# Autodesk Inventor assembly: MotorEsOrsoHajtas
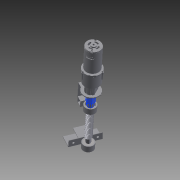
[picture p0: Inventor's stored thumbnail of the model, 180x180]
Saved by Autodesk Inventor 2015 SP1 (Build 190203100, 203)
## iProperties
Created: 2014-10-20
Part Number: MotorEsOrsoHajtas
Document SubType Name: Assembly
Designer: laca
Author: laca
## Documents named in this file (8)
- C:\Users\laca\Desktop\RobotMechanika\MotorEsOrsoHajtas.iam
- C:\Users\laca\Desktop\RobotMechanika\MotorTartoElso.ipt
- C:\Users\laca\Desktop\RobotMechanika\HatsoTartoJobb.ipt
- C:\Users\laca\Desktop\RobotMechanika\AnyaKicsi.ipt
- C:\Users\laca\Desktop\RobotMechanika\Csapagy6900.ipt
- C:\Users\laca\Desktop\RobotMechanika\Biztositek15mm.ipt
- C:\Users\laca\Desktop\RobotMechanika\Motor.iam
- C:\Users\laca\Desktop\RobotMechanika\Worm1.ipt
## Components (9 placed, 7 different names)
1. MotorTartoElso:1 — Rigid:1, Insert:5, Insert:6
2. HatsoTartoJobb:1 — Rotational:3
3. AnyaKicsi:1 — Rigid:3, Rigid:4, Cylindrical:7
4. Csapagy6900:1 — Rotational:3, Rigid:5
5. Csapagy6900:2 — Rigid:1, Cylindrical:6
6. Biztositek15mm:1 — Rigid:3, Cylindrical:5
7. Biztositek15mm:2 — Rigid:4, Cylindrical:4
8. Motor:1 [sub-assembly] — Insert:5, Cylindrical:4, Insert:6
9. Worm:2 — Rigid:5, Cylindrical:5, Cylindrical:6, Cylindrical:7
## Relationships (11: WeldJoint 4, CylindricalJoint 4, Insert 2, RevoluteJoint 1)
- Rotational:3 [RevoluteJoint]: HatsoTartoJobb:1 ↔ Csapagy6900:1
- Rigid:1 [WeldJoint]: MotorTartoElso:1 ↔ Csapagy6900:2
- Rigid:3 [WeldJoint]: AnyaKicsi:1 ↔ Biztositek15mm:1
- Rigid:4 [WeldJoint]: AnyaKicsi:1 ↔ Biztositek15mm:2
- Insert:5: MotorTartoElso:1 ↔ Motor:1
- Cylindrical:4: Biztositek15mm:2 ↔ Motor:1
- Insert:6: MotorTartoElso:1 ↔ Motor:1
- Rigid:5 [WeldJoint]: Csapagy6900:1 ↔ Worm:2
- Cylindrical:5: Biztositek15mm:1 ↔ Worm:2
- Cylindrical:6: Csapagy6900:2 ↔ Worm:2
- Cylindrical:7: AnyaKicsi:1 ↔ Worm:2
